# Autodesk Inventor assembly: Assembly1
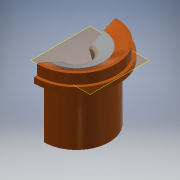
[picture p0: Inventor's stored thumbnail of the model, 180x180]
Saved by Autodesk Inventor 2017 (Build 210142000, 142)
## iProperties
Created: 2016-10-15
Part Number: Assembly1
Document SubType Name: Assembly
Designer: hyhe
Author: hyhe
## Documents named in this file (3)
- E:\Assembly1.iam
- C:\Users\hyhe\Downloads\Graphite Master Sketch.ipt
- C:\Users\hyhe\Downloads\Phenolic Master Sketch.ipt
## Components (2 placed, 2 different names)
1. Graphite Master Sketch:1 — Mate:1, Flush:1
2. Phenolic Master Sketch:1 — Mate:1
## Relationships (2: Mate 1, Flush 1)
- Mate:1: Graphite Master Sketch:1 ↔ Phenolic Master Sketch:1
- Flush:1: Graphite Master Sketch:1
